# Autodesk Inventor assembly: Propuesta_manufactura
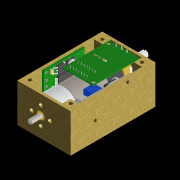
[picture p0: Inventor's stored thumbnail of the model, 180x180]
Saved by Autodesk Inventor 2020 (Build 240168000, 168)
## iProperties
Created: 2021-12-09
Part Number: Propuesta_manufactura
Document SubType Name: Assembly
Designer: juan
Author: juan
## Documents named in this file (7)
- C:\Users\juan\Documents\GitHub\Proyecto_de_Graduacion\Propuesta_manufactura\Popuesta_carcasa\Propuesta_manufactura.iam
- C:\Users\juan\Documents\GitHub\Proyecto_de_Graduacion\Propuesta_manufactura\Popuesta_carcasa\Parte de abajo contenedor.ipt
- C:\Users\juan\Documents\GitHub\Proyecto_de_Graduacion\Propuesta_manufactura\Popuesta_carcasa\25d-metal-gearmotor-20.4-encoder.ipt
- C:\Users\juan\Documents\GitHub\Proyecto_de_Graduacion\Propuesta_manufactura\Popuesta_carcasa\vnh5019-motor-driver-carrier.ipt
- C:\Users\juan\Documents\GitHub\Proyecto_de_Graduacion\Propuesta_manufactura\Popuesta_carcasa\LM2596 DC-DC StepDown Converter v1.ipt
- C:\Users\juan\Documents\GitHub\Proyecto_de_Graduacion\Propuesta_manufactura\Popuesta_carcasa\Tapadera_carcasa.ipt
- C:\Users\juan\Documents\GitHub\Proyecto_de_Graduacion\Propuesta_manufactura\Popuesta_carcasa\CONTROLADOR.ipt
## Components (6 placed, 6 different names)
1. Parte de abajo contenedor:1 — Mate:1, Mate:2, Mate:3, Mate:4, Mate:5, Mate:6, Mate:7, Mate:8, Flush:1, Flush:2, Mate:10, Mate:11
2. 25d-metal-gearmotor-20.4-encoder:1 — Mate:1, Mate:2, Mate:3
3. vnh5019-motor-driver-carrier:1 — Mate:4, Mate:5, Mate:6
4. LM2596 DC-DC StepDown Converter v1:1 — Mate:7, Mate:8
5. Tapadera_carcasa:1 — Flush:1, Flush:2, Mate:9
6. CONTROLADOR:1 — Mate:9, Mate:10, Mate:11
## Relationships (13: Mate 11, Flush 2)
- Mate:1: Parte de abajo contenedor:1 ↔ 25d-metal-gearmotor-20.4-encoder:1
- Mate:2: Parte de abajo contenedor:1 ↔ 25d-metal-gearmotor-20.4-encoder:1
- Mate:3: Parte de abajo contenedor:1 ↔ 25d-metal-gearmotor-20.4-encoder:1
- Mate:4: Parte de abajo contenedor:1 ↔ vnh5019-motor-driver-carrier:1
- Mate:5: Parte de abajo contenedor:1 ↔ vnh5019-motor-driver-carrier:1
- Mate:6: Parte de abajo contenedor:1 ↔ vnh5019-motor-driver-carrier:1
- Mate:7: Parte de abajo contenedor:1 ↔ LM2596 DC-DC StepDown Converter v1:1
- Mate:8: Parte de abajo contenedor:1 ↔ LM2596 DC-DC StepDown Converter v1:1
- Flush:1: Parte de abajo contenedor:1 ↔ Tapadera_carcasa:1
- Flush:2: Parte de abajo contenedor:1 ↔ Tapadera_carcasa:1
- Mate:9: Tapadera_carcasa:1 ↔ CONTROLADOR:1
- Mate:10: Parte de abajo contenedor:1 ↔ CONTROLADOR:1
- Mate:11: Parte de abajo contenedor:1 ↔ CONTROLADOR:1
